# Autodesk Inventor assembly: Joint Assembly
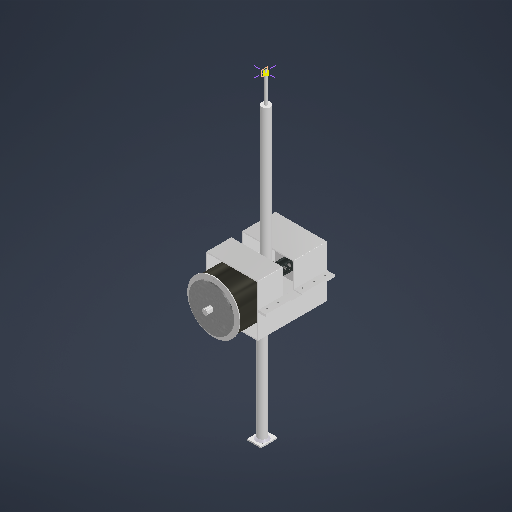
[picture p0: Inventor's stored thumbnail of the model, 512x512]
Saved by Autodesk Inventor 2026.3 (Build 303398000, 398)
## iProperties
Created: 2026-07-22
Part Number: Joint Assembly
Document SubType Name: Assembly
Designer: matot
Author: matot
## Documents named in this file (18)
- C:\Users\matot\OneDrive - Stellenbosch University\2026\MechatronicsProject478\Building the joint\Joint Assembly\Joint Assembly.iam
- C:\Users\matot\OneDrive - Stellenbosch University\2026\MechatronicsProject478\Building the joint\Joint Assembly\2058786.iam
- C:\Users\matot\OneDrive - Stellenbosch University\2026\MechatronicsProject478\Building the joint\Joint Assembly\Reducer bushing.ipt
- C:\Users\matot\OneDrive - Stellenbosch University\2026\MechatronicsProject478\Building the joint\Joint Assembly\Optical Encoder.ipt
- C:\Users\matot\OneDrive - Stellenbosch University\2026\MechatronicsProject478\Building the joint\Joint Assembly\Rough draft shaft.ipt
- C:\Users\matot\OneDrive - Stellenbosch University\2026\MechatronicsProject478\Building the joint\Joint Assembly\8236976.ipt
- C:\Users\matot\OneDrive - Stellenbosch University\2026\MechatronicsProject478\Building the joint\Joint Assembly\mclx-20-20-f.iam
- C:\Users\matot\OneDrive - Stellenbosch University\2026\MechatronicsProject478\Building the joint\Joint Assembly\Electromagnet.iam
- C:\Users\matot\OneDrive - Stellenbosch University\2026\MechatronicsProject478\Building the joint\Joint Assembly\Prressure plate.ipt
- C:\Users\matot\OneDrive - Stellenbosch University\2026\MechatronicsProject478\Building the joint\Joint Assembly\Friction Plate.ipt
- C:\Users\matot\OneDrive - Stellenbosch University\2026\MechatronicsProject478\Building the joint\Joint Assembly\Brake disc.ipt
- C:\Users\matot\OneDrive - Stellenbosch University\2026\MechatronicsProject478\Building the joint\Joint Assembly\Joint Housing Bottom.iam
- C:\Users\matot\OneDrive - Stellenbosch University\2026\MechatronicsProject478\Building the joint\Joint Assembly\Bearing housing top.ipt
- C:\Users\matot\OneDrive - Stellenbosch University\2026\MechatronicsProject478\Building the joint\Joint Assembly\Bearing housing bottom.ipt
- C:\Users\matot\OneDrive - Stellenbosch University\2026\MechatronicsProject478\Building the joint\Joint Assembly\Output Link.iam
- C:\Users\matot\OneDrive - Stellenbosch University\2026\MechatronicsProject478\Building the joint\Joint Assembly\Base link.iam
- C:\Users\matot\OneDrive - Stellenbosch University\2026\MechatronicsProject478\Building the joint\Joint Assembly\Top joint housing.ipt
- C:\Users\matot\OneDrive - Stellenbosch University\2026\MechatronicsProject478\Building the joint\Joint Assembly\Top joint housing back.iam
## Components (21 placed, 17 different names)
1. Rough draft shaft:1 — Insert:1, Insert:2, Mate:1
2. 2058786:1 [sub-assembly] — Insert:1, Insert:4, Insert:14, Insert:16
3. 2058786:2 [sub-assembly] — Insert:2, Insert:3, Insert:13, Insert:15
4. 8236976:3 — Insert:3, Insert:8
5. 8236976:4 — Insert:4, Insert:7
6. Optical Encoder:1 — Insert:5, Insert:6
7. Reducer bushing:1 — Insert:5
8. mclx-20-20-f:1 [sub-assembly] — Insert:6, Insert:7
9. Electromagnet:1 [sub-assembly] — Insert:8, Insert:9, Insert:10, Tangent:1, Tangent:2
10. Prressure plate:1 — Insert:9, Insert:10, Insert:11
11. Friction Plate:1 — Insert:11, Insert:12
12. Brake disc:1 — Insert:12
13. Joint Housing Bottom:1 [sub-assembly] — Tangent:1, Tangent:2, Insert:17, Insert:18, Mate:2, Flush:1, Flush:2, Mate:3, Flush:3, Flush:4
14. Bearing housing top:3 — Insert:13
15. Bearing housing top:4 — Insert:14
16. Bearing housing bottom:1 — Insert:15, Insert:17
17. Bearing housing bottom:2 — Insert:16
18. Output Link:1 [sub-assembly] — Mate:1
19. Base link:1 [sub-assembly] — Insert:18
20. Top joint housing:1 — Mate:2, Flush:1, Flush:2
21. Top joint housing back:1 [sub-assembly] — Mate:3, Flush:3, Flush:4
## Relationships (27: Insert 18, Flush 4, Mate 3, Tangent 2)
- Insert:1: Rough draft shaft:1 ↔ 2058786:1
- Insert:2: Rough draft shaft:1 ↔ 2058786:2
- Insert:3: 2058786:2 ↔ 8236976:3
- Insert:4: 2058786:1 ↔ 8236976:4
- Insert:5: Optical Encoder:1 ↔ Reducer bushing:1
- Insert:6: Optical Encoder:1 ↔ mclx-20-20-f:1
- Insert:7: 8236976:4 ↔ mclx-20-20-f:1
- Insert:8: 8236976:3 ↔ Electromagnet:1
- Insert:9: Electromagnet:1 ↔ Prressure plate:1
- Insert:10: Electromagnet:1 ↔ Prressure plate:1
- Insert:11: Prressure plate:1 ↔ Friction Plate:1
- Insert:12: Friction Plate:1 ↔ Brake disc:1
- Tangent:1: Electromagnet:1 ↔ Joint Housing Bottom:1
- Tangent:2: Electromagnet:1 ↔ Joint Housing Bottom:1
- Insert:13: 2058786:2 ↔ Bearing housing top:3
- Insert:14: 2058786:1 ↔ Bearing housing top:4
- Insert:15: 2058786:2 ↔ Bearing housing bottom:1
- Insert:16: 2058786:1 ↔ Bearing housing bottom:2
- Insert:17: Joint Housing Bottom:1 ↔ Bearing housing bottom:1
- Mate:1: Rough draft shaft:1 ↔ Output Link:1
- Insert:18: Joint Housing Bottom:1 ↔ Base link:1
- Mate:2: Joint Housing Bottom:1 ↔ Top joint housing:1
- Flush:1: Joint Housing Bottom:1 ↔ Top joint housing:1
- Flush:2: Joint Housing Bottom:1 ↔ Top joint housing:1
- Mate:3: Joint Housing Bottom:1 ↔ Top joint housing back:1
- Flush:3: Joint Housing Bottom:1 ↔ Top joint housing back:1
- Flush:4: Joint Housing Bottom:1 ↔ Top joint housing back:1
